# Autodesk Inventor assembly: GripCharger
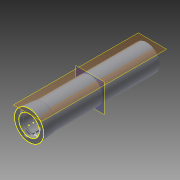
[picture p0: Inventor's stored thumbnail of the model, 180x180]
Saved by Autodesk Inventor 2014 SP1 (Build 180222100, 222)
## iProperties
Created: 2015-10-17
Part Number: GripCharger
Document SubType Name: Assembly
Designer: anthony
Author: anthony
## Documents named in this file (3)
- C:\Users\anthony\Documents\HardwareHack\GripCharger.iam
- C:\Users\anthony\Documents\HardwareHack\GripOuterTube.ipt
- C:\Users\anthony\Documents\HardwareHack\GripScrewCap.ipt
## Components (2 placed, 2 different names)
1. GripOuterTube:1 — Rotational:1
2. GripScrewCap:1 — Rotational:1
## Relationships (1: RevoluteJoint 1)
- Rotational:1 [RevoluteJoint]: GripOuterTube:1 ↔ GripScrewCap:1
